# Autodesk Inventor assembly: Tank tread with rubber insert
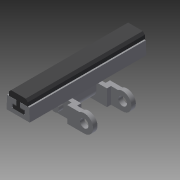
[picture p0: Inventor's stored thumbnail of the model, 180x180]
Saved by Autodesk Inventor 2015 (Build 190159000, 159)
## iProperties
Created: 2015-09-30
Part Number: Tank tread with rubber insert
Document SubType Name: Assembly
Designer: alhohbein
Author: alhohbein
## Documents named in this file (3)
- C:\Users\alhohbein\Documents\Tank tread with rubber insert.iam
- U:\TETRIX_736468_TT_LINK_2012.ipt
- U:\TETRIX_736468_TT_INSERT_2012.ipt
## Components (2 placed, 2 different names)
1. TETRIX_736468_TT_LINK_2012:1 — Mate:1, Flush:1, Mate:2
2. TETRIX_736468_TT_INSERT_2012:1 — Mate:1, Flush:1, Mate:2
## Relationships (3: Mate 2, Flush 1)
- Mate:1: TETRIX_736468_TT_LINK_2012:1 ↔ TETRIX_736468_TT_INSERT_2012:1
- Flush:1: TETRIX_736468_TT_LINK_2012:1 ↔ TETRIX_736468_TT_INSERT_2012:1
- Mate:2: TETRIX_736468_TT_LINK_2012:1 ↔ TETRIX_736468_TT_INSERT_2012:1
